# Autodesk Inventor assembly: roka
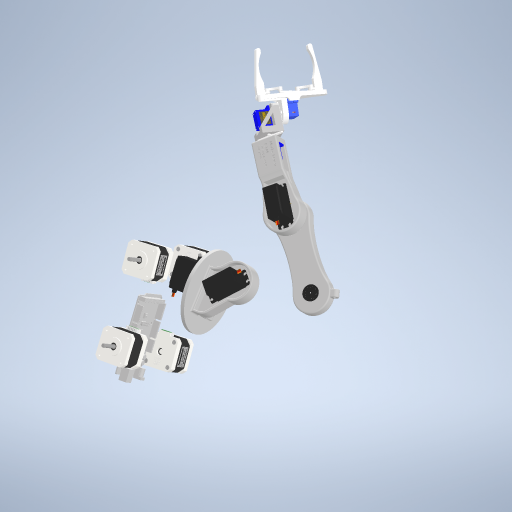
[picture p0: Inventor's stored thumbnail of the model, 512x512]
Saved by Autodesk Inventor 2024 (Build 280153000, 153)
## iProperties
Created: 2023-09-17
Part Number: roka
Document SubType Name: Assembly
Designer: jebes windows
Author: jebes windows
## Documents named in this file (14)
- C:\Users\jebes windows\Documents\Inventor\Robotska_roka\roka.iam
- C:\Users\jebes windows\Documents\Inventor\Robotska_roka\vozicek1.ipt
- C:\Users\jebes windows\Documents\Inventor\Robotska_roka\Nema 17 Motor a Pasos 17HS4401\Nema 17 Motor a Pasos 17HS4401.ipt
- C:\Users\jebes windows\Documents\Inventor\Robotska_roka\ArduinoMega_STEP_AP203\ArduinoMega_STEP_AP203.ipt
- C:\Users\jebes windows\Documents\Inventor\Robotska_roka\servo-motor-mg996r-1.snapshot.1(2)\Servo Motor MG996R  With Attachments\Servo Motor MG996R  With Attachments.iam
- C:\Users\jebes windows\Documents\Inventor\Robotska_roka\miza.ipt
- C:\Users\jebes windows\Documents\Inventor\Robotska_roka\pokrow.ipt
- C:\Users\jebes windows\Documents\Inventor\Robotska_roka\roka1.ipt
- C:\Users\jebes windows\Documents\Inventor\Robotska_roka\roka2.ipt
- C:\Users\jebes windows\Documents\Inventor\Robotska_roka\sg90-micro-servo-9g-tower-pro-1.snapshot.3\SG90 - Micro Servo 9g - Tower Pro\SG90 - Micro Servo 9g - Tower Pro.iam
- C:\Users\jebes windows\Documents\Inventor\Robotska_roka\roka3.ipt
- E:\dowloads\gewiss-gw-44-207-enclosure-1.snapshot.1\GW44207\GW44207 ENCLOSURE.iam
- C:\Users\jebes windows\Documents\Inventor\Robotska_roka\adasd.ipt
- C:\Users\jebes windows\Documents\Inventor\Robotska_roka\linear-gripper-1.snapshot.4\Linear Gripper\GRIPPER.iam
## Components (23 placed, 13 different names)
1. vozicek:1 — Rigid:8
2. Nema 17 Motor a Pasos 17HS4401:1 — Insert:2, Flush:3
3. Nema 17 Motor a Pasos 17HS4401:2 — Insert:4
4. Nema 17 Motor a Pasos 17HS4401:3 — Insert:3
5. Nema 17 Motor a Pasos 17HS4401:4 — Insert:1, Rotational:10
6. ArduinoMega_STEP_AP203:1 — Mate:1, Mate:2
7. Servo Motor MG996R  With Attachments:1 [sub-assembly] — Rotational:1, Rotational:11
8. Servo Motor MG996R  With Attachments:2 [sub-assembly] — Rotational:1, Rigid:7
9. miza:1 — Rigid:7, Flush:2, Rotational:13
10. pokrow:1 — Rigid:8
11. Servo Motor MG996R  With Attachments:3 [sub-assembly] — Rotational:13
12. Servo Motor MG996R  With Attachments:4 [sub-assembly] — Rotational:3, Angle:1
13. roka1:1 — Rotational:3, Rotational:5, Flush:2
14. roka2:1 — Rigid:10, Rigid:11
15. Servo Motor MG996R  With Attachments:5 [sub-assembly] — Rigid:10
16. Servo Motor MG996R  With Attachments:6 [sub-assembly] — Rotational:5
17. SG90 - Micro Servo 9g - Tower Pro:1 [sub-assembly] — Rigid:11, Rotational:6
18. SG90 - Micro Servo 9g - Tower Pro:3 [sub-assembly] — Rigid:13, Rotational:12
19. roka3:1 — Rigid:13, Rotational:6
20. GW44207 ENCLOSURE:1 [sub-assembly] — Insert:1, Insert:2, Insert:3, Insert:4, Mate:1, Mate:2, Rotational:11
21. adasd:1 — Flush:3
22. adasd:2 — Rotational:10
23. GRIPPER:1 [sub-assembly] — Rotational:12
## Relationships (23: RevoluteJoint 9, WeldJoint 5, Insert 4, Flush 2, Mate 2, Angle 1)
- Rotational:1 [RevoluteJoint]: Servo Motor MG996R  With Attachments:1 ↔ Servo Motor MG996R  With Attachments:2
- Rigid:7 [WeldJoint]: Servo Motor MG996R  With Attachments:2 ↔ miza:1
- Rigid:8 [WeldJoint]: vozicek:1 ↔ pokrow:1
- Rotational:3 [RevoluteJoint]: Servo Motor MG996R  With Attachments:4 ↔ roka1:1
- [RevoluteJoint]: Servo Motor MG996R  With Attachments:5 ↔ Servo Motor MG996R  With Attachments:6
- Rigid:10 [WeldJoint]: roka2:1 ↔ Servo Motor MG996R  With Attachments:5
- Rotational:5 [RevoluteJoint]: roka1:1 ↔ Servo Motor MG996R  With Attachments:6
- Rigid:11 [WeldJoint]: roka2:1 ↔ SG90 - Micro Servo 9g - Tower Pro:1
- Rigid:13 [WeldJoint]: SG90 - Micro Servo 9g - Tower Pro:3 ↔ roka3:1
- Rotational:6 [RevoluteJoint]: SG90 - Micro Servo 9g - Tower Pro:1 ↔ roka3:1
- Flush:2: miza:1 ↔ roka1:1
- Angle:1 (0 deg): Servo Motor MG996R  With Attachments:4
- Insert:1: Nema 17 Motor a Pasos 17HS4401:4 ↔ GW44207 ENCLOSURE:1
- Insert:2: Nema 17 Motor a Pasos 17HS4401:1 ↔ GW44207 ENCLOSURE:1
- Insert:3: Nema 17 Motor a Pasos 17HS4401:3 ↔ GW44207 ENCLOSURE:1
- Insert:4: Nema 17 Motor a Pasos 17HS4401:2 ↔ GW44207 ENCLOSURE:1
- Mate:1: ArduinoMega_STEP_AP203:1 ↔ GW44207 ENCLOSURE:1
- Mate:2: ArduinoMega_STEP_AP203:1 ↔ GW44207 ENCLOSURE:1
- Flush:3: Nema 17 Motor a Pasos 17HS4401:1 ↔ adasd:1
- Rotational:10 [RevoluteJoint]: Nema 17 Motor a Pasos 17HS4401:4 ↔ adasd:2
- Rotational:11 [RevoluteJoint]: Servo Motor MG996R  With Attachments:1 ↔ GW44207 ENCLOSURE:1
- Rotational:12 [RevoluteJoint]: SG90 - Micro Servo 9g - Tower Pro:3 ↔ GRIPPER:1
- Rotational:13 [RevoluteJoint]: miza:1 ↔ Servo Motor MG996R  With Attachments:3
## Named parameters: d15_d11 = 0 mm, d16_d12 = 68.17376 deg
